# Autodesk Inventor assembly: dmc_assembly
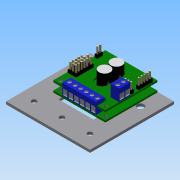
[picture p0: Inventor's stored thumbnail of the model, 180x180]
Saved by Autodesk Inventor 2015 (Build 190159000, 159)
## iProperties
Created: 2014-12-13
Part Number: dmc_assembly
Document SubType Name: Assembly
Designer: Daniel
Author: Daniel
## Documents named in this file (3)
- C:\Users\Daniel\Dropbox\Inventor\biscuitbot\dmc_assembly.iam
- C:\Users\Daniel\Dropbox\Inventor\biscuitbot\dmc_plate.ipt
- C:\Users\Daniel\Dropbox\Inventor\biscuitbot\Pololu_DMC01.ipt
## Components (2 placed, 2 different names)
1. dmc_plate:1 — Insert:1, Insert:2
2. Pololu_DMC01:1 — Insert:1, Insert:2
## Relationships (2: Insert 2)
- Insert:1: dmc_plate:1 ↔ Pololu_DMC01:1
- Insert:2: dmc_plate:1 ↔ Pololu_DMC01:1
